# Autodesk Inventor assembly: xl_wheel_ass
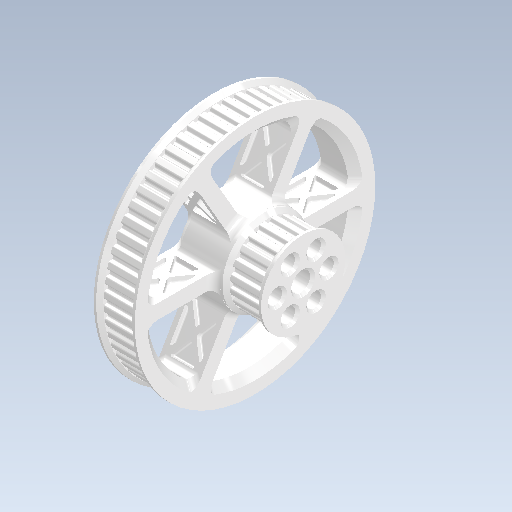
[picture p0: Inventor's stored thumbnail of the model, 512x512]
Saved by Autodesk Inventor 2020 (Build 240168000, 168)
## iProperties
Created: 2020-05-08
Part Number: xl_wheel_ass
Document SubType Name: Assembly
Designer: psrobotics
Author: psrobotics
## Documents named in this file (3)
- D:\projects-3\biped_gen1\hardware\xl_wheel_ass.iam
- D:\projects-3\biped_gen1\hardware\xl_60_ori.ipt
- D:\projects-3\biped_gen1\hardware\xl_20_ori.ipt
## Components (2 placed, 2 different names)
1. xl_60_ori:1 — Insert:2, Insert:3
2. xl_20_ori:1 — Insert:2, Insert:3
## Relationships (2: Insert 2)
- Insert:2: xl_60_ori:1 ↔ xl_20_ori:1
- Insert:3: xl_60_ori:1 ↔ xl_20_ori:1
